# Autodesk Inventor assembly: ArcadeBoxAssembly
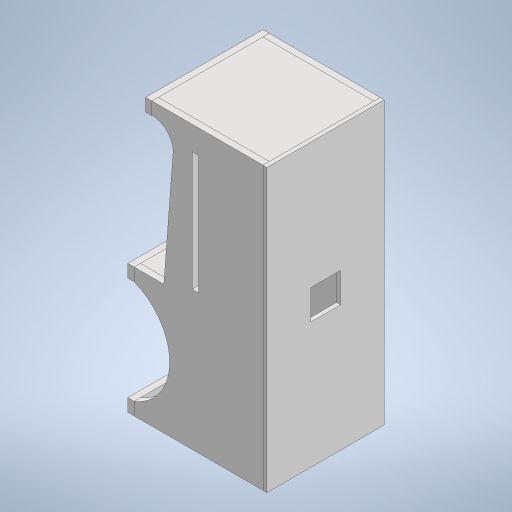
[picture p0: Inventor's stored thumbnail of the model, 512x512]
Saved by Autodesk Inventor 2024 (Build 280153000, 153)
## iProperties
Created: 2023-10-07
Part Number: ArcadeBoxAssembly
Document SubType Name: Assembly
Designer: chris
Author: chris
## Documents named in this file (10)
- C:\Users\chris\Documents\DIGITAL2\prueba\ArcadeBox\ArcadeBoxAssembly.iam
- C:\Users\chris\Documents\DIGITAL2\prueba\ArcadeBox\Base.ipt
- C:\Users\chris\Documents\DIGITAL2\prueba\ArcadeBox\LCD9341.ipt
- C:\Users\chris\Documents\DIGITAL2\prueba\ArcadeBox\LCDFrame.ipt
- C:\Users\chris\Documents\DIGITAL2\prueba\ArcadeBox\SideSupports.ipt
- C:\Users\chris\Documents\DIGITAL2\prueba\ArcadeBox\Decal.ipt
- C:\Users\chris\Documents\DIGITAL2\prueba\ArcadeBox\Base - Copy.ipt
- C:\Users\chris\Documents\DIGITAL2\prueba\ArcadeBox\BaseTop.ipt
- C:\Users\chris\Documents\DIGITAL2\prueba\ArcadeBox\Back.ipt
- C:\Users\chris\Documents\DIGITAL2\prueba\ArcadeBox\Front.ipt
## Components (12 placed, 9 different names)
1. LCD9341:1 — Mate:1, Mate:2, Mate:3
2. LCDFrame:1 — Mate:1, Mate:2, Mate:3, Mate:14, Mate:16, Mate:17, Flush:20
3. SideSupports:1 — Flush:7, Mate:15, Mate:21, Flush:16, Mate:22, Mate:24, Mate:26
4. SideSupports:2 — Mate:9, Flush:10, Flush:11, Mate:12, Mate:13, Mate:14, Mate:16, Mate:18, Flush:14, Flush:15, Mate:19, Mate:20, Flush:17, Flush:18, Flush:21, Flush:23
5. Base:3 — Flush:7, Mate:9, Mate:11, Flush:9, Mate:17, Flush:20, Flush:24
6. Decal:1 — Flush:11, Mate:13, Flush:19
7. Decal:2 — Mate:11, Flush:9, Flush:10, Mate:12, Mate:15
8. Decal:3 — Mate:18, Flush:14, Flush:15, Mate:23
9. Base - Copy:1 — Mate:19, Mate:20, Mate:21, Flush:16, Flush:17, Flush:18, Flush:19, Mate:25
10. BaseTop:1 — Mate:22, Flush:21, Mate:23, Flush:22
11. Back:1 — Mate:24, Flush:22, Flush:23
12. Front:1 — Mate:25, Mate:26, Flush:24
## Relationships (35: Mate 20, Flush 15)
- Mate:1: LCD9341:1 ↔ LCDFrame:1
- Mate:2: LCD9341:1 ↔ LCDFrame:1
- Mate:3 (0.7 mm): LCD9341:1 ↔ LCDFrame:1
- Flush:7: SideSupports:1 ↔ Base:3
- Mate:9: SideSupports:2 ↔ Base:3
- Mate:11: Base:3 ↔ Decal:2
- Flush:9: Base:3 ↔ Decal:2
- Flush:10: SideSupports:2 ↔ Decal:2
- Flush:11: SideSupports:2 ↔ Decal:1
- Mate:12: SideSupports:2 ↔ Decal:2
- Mate:13: SideSupports:2 ↔ Decal:1
- Mate:14: LCDFrame:1 ↔ SideSupports:2
- Mate:15: SideSupports:1 ↔ Decal:2
- Mate:16: LCDFrame:1 ↔ SideSupports:2
- Mate:17: LCDFrame:1 ↔ Base:3
- Mate:18: SideSupports:2 ↔ Decal:3
- Flush:14: SideSupports:2 ↔ Decal:3
- Flush:15: SideSupports:2 ↔ Decal:3
- Mate:19: SideSupports:2 ↔ Base - Copy:1
- Mate:20: SideSupports:2 ↔ Base - Copy:1
- Mate:21: SideSupports:1 ↔ Base - Copy:1
- Flush:16: SideSupports:1 ↔ Base - Copy:1
- Flush:17: SideSupports:2 ↔ Base - Copy:1
- Flush:18: SideSupports:2 ↔ Base - Copy:1
- Flush:19: Decal:1 ↔ Base - Copy:1
- Flush:20: LCDFrame:1 ↔ Base:3
- Mate:22: SideSupports:1 ↔ BaseTop:1
- Flush:21: SideSupports:2 ↔ BaseTop:1
- Mate:23: Decal:3 ↔ BaseTop:1
- Mate:24: SideSupports:1 ↔ Back:1
- Flush:22: BaseTop:1 ↔ Back:1
- Flush:23: SideSupports:2 ↔ Back:1
- Mate:25: Base - Copy:1 ↔ Front:1
- Mate:26: SideSupports:1 ↔ Front:1
- Flush:24: Base:3 ↔ Front:1
